# Autodesk Inventor assembly: 垃圾桶上层
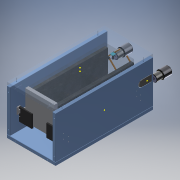
[picture p0: Inventor's stored thumbnail of the model, 180x180]
Saved by Autodesk Inventor 2017 (Build 210142000, 142)
## iProperties
Part Number: 垃圾桶上层
Material: 常规
Document SubType Name: Assembly
Designer: PANDA
Author: PANDA
## Documents named in this file (15)
- D:\PANDA\Study\VG100\P2\草图\垃圾桶丝轴滑杆\垃圾桶上层.iam
- D:\PANDA\Study\VG100\P2\草图\垃圾桶丝轴滑杆\垃圾桶正版.ipt
- D:\PANDA\Study\VG100\P2\草图\垃圾桶丝轴滑杆\垃圾桶侧板.ipt
- D:\PANDA\Study\VG100\P2\草图\垃圾桶丝轴滑杆\马达.ipt
- D:\PANDA\Study\VG100\P2\草图\垃圾桶丝轴滑杆\激光传感器.ipt
- D:\PANDA\Study\VG100\P2\草图\垃圾桶丝轴滑杆\内层升降板.ipt
- D:\PANDA\Study\VG100\P2\草图\垃圾桶丝轴滑杆\内层正板.ipt
- D:\PANDA\Study\VG100\P2\草图\垃圾桶丝轴滑杆\内层侧板.ipt
- D:\PANDA\Study\VG100\P2\草图\垃圾桶丝轴滑杆\推杆电机.ipt
- D:\PANDA\Study\VG100\P2\草图\垃圾桶丝轴滑杆\打包支架.ipt
- D:\PANDA\Study\VG100\P2\草图\垃圾桶丝轴滑杆\压缩杆.ipt
- D:\PANDA\Study\VG100\P2\草图\垃圾桶丝轴滑杆\滑竿固定器.ipt
- D:\PANDA\Study\VG100\P2\草图\垃圾桶丝轴滑杆\长轴.ipt
- D:\PANDA\Study\VG100\P2\草图\垃圾桶丝轴滑杆\丝杆.ipt
- D:\PANDA\Study\VG100\P2\草图\垃圾桶丝轴滑杆\升降板.ipt
## Components (33 placed, 14 different names)
1. 垃圾桶正版:1 — 旋转:3, 旋转:7
2. 垃圾桶侧板:2 — 旋转:3, 旋转:4, 旋转:5, 刚性:22, 旋转:67, 旋转:68, 旋转:70, 旋转:81
3. 垃圾桶正版:2 — 旋转:4, 旋转:5, 旋转:6
4. 垃圾桶侧板:3 — 旋转:6, 旋转:7, 旋转:58, 旋转:63, 旋转:64, 旋转:65, 旋转:78
5. 内层升降板:1 — 旋转:44, 旋转:45, 旋转:46, 旋转:47, 旋转:48
6. 内层正板:1 — 旋转:44, 旋转:57
7. 内层正板:2 — 旋转:45, 刚性:20
8. 内层侧板:1 — 旋转:46
9. 内层侧板:2 — 旋转:47, 旋转:48
10. 激光传感器:3 — 刚性:20
11. 激光传感器:4 — 旋转:57
12. 推杆电机:1 — 旋转:58, 旋转:60
13. 打包支架:1 — 旋转:59, 旋转:62
14. 打包支架:2 — 旋转:60, 旋转:61
15. 推杆电机:2 — 刚性:22, 旋转:59
16. 压缩杆:1 — 旋转:61
17. 压缩杆:2 — 旋转:62
18. 滑竿固定器:1 — 旋转:63, 刚性:23
19. 滑竿固定器:2 — 旋转:67, 旋转:77
20. 滑竿固定器:3 — 旋转:64
21. 滑竿固定器:4 — 旋转:65
22. 滑竿固定器:6 — 旋转:70
23. 滑竿固定器:8 — 旋转:68
24. 丝杆:1 — 旋转:77, 刚性:24
25. 丝杆:2 — 刚性:23, 旋转:85
26. 滑竿固定器:9 — 旋转:78, 旋转:80
27. 长轴:1 — 旋转:80, 旋转:84
28. 马达:5 — 旋转:83
29. 马达:6 — 旋转:84
30. 滑竿固定器:10 — 旋转:81, 旋转:82
31. 长轴:2 — 旋转:82, 旋转:83
32. 升降板:2 — 刚性:24
33. 升降板:3 — 旋转:85
## Relationships (34: RevoluteJoint 30, WeldJoint 4)
- 旋转:3 [RevoluteJoint]: 垃圾桶正版:1 ↔ 垃圾桶侧板:2
- 旋转:4 [RevoluteJoint]: 垃圾桶侧板:2 ↔ 垃圾桶正版:2
- 旋转:5 [RevoluteJoint]: 垃圾桶侧板:2 ↔ 垃圾桶正版:2
- 旋转:6 [RevoluteJoint]: 垃圾桶正版:2 ↔ 垃圾桶侧板:3
- 旋转:7 [RevoluteJoint]: 垃圾桶正版:1 ↔ 垃圾桶侧板:3
- 旋转:44 [RevoluteJoint]: 内层升降板:1 ↔ 内层正板:1
- 旋转:45 [RevoluteJoint]: 内层升降板:1 ↔ 内层正板:2
- 旋转:46 [RevoluteJoint]: 内层升降板:1 ↔ 内层侧板:1
- 旋转:47 [RevoluteJoint]: 内层升降板:1 ↔ 内层侧板:2
- 旋转:48 [RevoluteJoint]: 内层升降板:1 ↔ 内层侧板:2
- 刚性:20 [WeldJoint]: 内层正板:2 ↔ 激光传感器:3
- 旋转:57 [RevoluteJoint]: 内层正板:1 ↔ 激光传感器:4
- 旋转:58 [RevoluteJoint]: 垃圾桶侧板:3 ↔ 推杆电机:1
- 刚性:22 [WeldJoint]: 垃圾桶侧板:2 ↔ 推杆电机:2
- 旋转:59 [RevoluteJoint]: 打包支架:1 ↔ 推杆电机:2
- 旋转:60 [RevoluteJoint]: 推杆电机:1 ↔ 打包支架:2
- 旋转:61 [RevoluteJoint]: 打包支架:2 ↔ 压缩杆:1
- 旋转:62 [RevoluteJoint]: 打包支架:1 ↔ 压缩杆:2
- 旋转:63 [RevoluteJoint]: 垃圾桶侧板:3 ↔ 滑竿固定器:1
- 旋转:64 [RevoluteJoint]: 垃圾桶侧板:3 ↔ 滑竿固定器:3
- 旋转:65 [RevoluteJoint]: 垃圾桶侧板:3 ↔ 滑竿固定器:4
- 旋转:67 [RevoluteJoint]: 垃圾桶侧板:2 ↔ 滑竿固定器:2
- 旋转:68 [RevoluteJoint]: 垃圾桶侧板:2 ↔ 滑竿固定器:8
- 旋转:70 [RevoluteJoint]: 垃圾桶侧板:2 ↔ 滑竿固定器:6
- 旋转:77 [RevoluteJoint]: 滑竿固定器:2 ↔ 丝杆:1
- 刚性:23 [WeldJoint]: 滑竿固定器:1 ↔ 丝杆:2
- 旋转:78 [RevoluteJoint]: 垃圾桶侧板:3 ↔ 滑竿固定器:9
- 旋转:80 [RevoluteJoint]: 滑竿固定器:9 ↔ 长轴:1
- 旋转:81 [RevoluteJoint]: 垃圾桶侧板:2 ↔ 滑竿固定器:10
- 旋转:82 [RevoluteJoint]: 滑竿固定器:10 ↔ 长轴:2
- 旋转:83 [RevoluteJoint]: 马达:5 ↔ 长轴:2
- 旋转:84 [RevoluteJoint]: 长轴:1 ↔ 马达:6
- 刚性:24 [WeldJoint]: 丝杆:1 ↔ 升降板:2
- 旋转:85 [RevoluteJoint]: 丝杆:2 ↔ 升降板:3
